# Autodesk Inventor assembly: Leadscrew Bearing Assembly
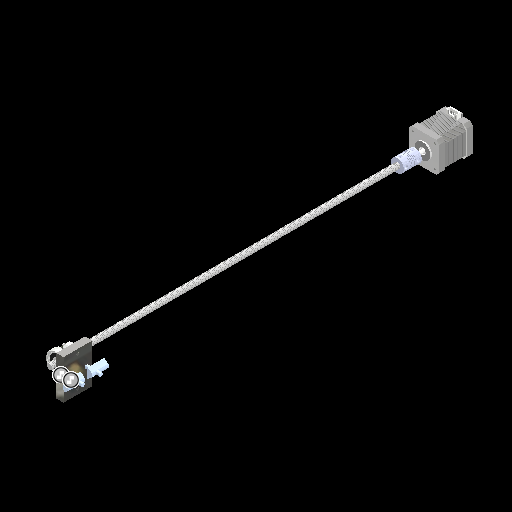
[picture p0: Inventor's stored thumbnail of the model, 512x512]
Saved by Autodesk Inventor 2026.1 (Build 301233000, 233)
## iProperties
Created: 2024-12-30
Part Number: Leadscrew Bearing Assembly
Document SubType Name: Assembly
Designer: drago
Author: drago
## Documents named in this file (9)
- C:\Users\drago\Desktop\_QIST4500_Multidisciplinary_Team_Project\Proteox MX magnet positioner CAD\magnet_positioner_cad_design\z_translator\z_translator.iam
- C:\Users\drago\Desktop\_QIST4500_Multidisciplinary_Team_Project\Proteox MX magnet positioner CAD\magnet_positioner_cad_design\z_translator\5X8_COUPLER.ipt
- C:\Users\drago\Desktop\_QIST4500_Multidisciplinary_Team_Project\Proteox MX magnet positioner CAD\magnet_positioner_cad_design\z_translator\item_61953_t-slot-slider-8-80x40-fa__high.ipt
- C:\Users\drago\Desktop\_QIST4500_Multidisciplinary_Team_Project\Proteox MX magnet positioner CAD\magnet_positioner_cad_design\z_translator\KP08.iam
- C:\Users\drago\Desktop\_QIST4500_Multidisciplinary_Team_Project\Proteox MX magnet positioner CAD\magnet_positioner_cad_design\z_translator\Leadscrew Bearing Bracket.ipt
- C:\Users\drago\Desktop\_QIST4500_Multidisciplinary_Team_Project\Proteox MX magnet positioner CAD\magnet_positioner_cad_design\z_translator\Lead Screw 8mm-2.0 x 500mm.ipt
- C:\Users\drago\Desktop\_QIST4500_Multidisciplinary_Team_Project\Proteox MX magnet positioner CAD\magnet_positioner_cad_design\z_translator\Stepper Motor Nema 17.ipt
- C:\Users\drago\Documents\Inventor\Content Center Files\R2026\en-US\ISO 7089\ISO 7089 - 4 - 140 HV(1).ipt
- C:\Users\drago\Documents\Inventor\Content Center Files\R2026\en-US\ISO 4762(2)\ISO 4762 - M4 x 16ISO.ipt
## Components (11 placed, 8 different names)
1. 5X8_COUPLER:1 — Mate:11, Mate:14, Mate:16, Mate:20
2. item_61953_t-slot-slider-8-80x40-fa__high:1 — Angle:3, Mate:21, Mate:23
3. item_61953_t-slot-slider-8-80x40-fa__high:2 — Angle:2, Mate:22, Mate:24
4. KP08:1 [sub-assembly] — Mate:12, Mate:13, Mate:25, Mate:26, Mate:27, Mate:29, Mate:31
5. Leadscrew Bearing Bracket:1 — Mate:21, Mate:22, Mate:23, Mate:24, Mate:25, Mate:26, Mate:27, Angle:4, Mate:28, Mate:30
6. Lead Screw 8mm-2.0 x 500mm:1 — Mate:11, Mate:12, Mate:13, Mate:15, Mate:19
7. Stepper Motor Nema 17:1 — Mate:14, Mate:15, Mate:16, Mate:17, Mate:18
8. ISO 4762 M4 x 16:2 — Insert:2
9. ISO 7089 4:2 — Mate:30, Mate:31, Insert:2
10. ISO 4762 M4 x 16:1 — Insert:1
11. ISO 7089 4:1 — Mate:28, Mate:29, Insert:1
## Relationships (26: Mate 21, Angle 3, Insert 2)
- Mate:11: 5X8_COUPLER:1 ↔ Lead Screw 8mm-2.0 x 500mm:1
- Mate:12: KP08:1 ↔ Lead Screw 8mm-2.0 x 500mm:1
- Mate:13 (-10 mm): KP08:1 ↔ Lead Screw 8mm-2.0 x 500mm:1
- Mate:14: 5X8_COUPLER:1 ↔ Stepper Motor Nema 17:1
- Mate:15: Lead Screw 8mm-2.0 x 500mm:1 ↔ Stepper Motor Nema 17:1
- Mate:16 (10 mm): 5X8_COUPLER:1 ↔ Stepper Motor Nema 17:1
- Mate:17: Stepper Motor Nema 17:1
- Mate:18: Stepper Motor Nema 17:1
- Mate:19: Lead Screw 8mm-2.0 x 500mm:1
- Angle:2 (0 deg): item_61953_t-slot-slider-8-80x40-fa__high:2
- Angle:3 (180 deg): item_61953_t-slot-slider-8-80x40-fa__high:1
- Mate:20: 5X8_COUPLER:1
- Mate:21: item_61953_t-slot-slider-8-80x40-fa__high:1 ↔ Leadscrew Bearing Bracket:1
- Mate:22: item_61953_t-slot-slider-8-80x40-fa__high:2 ↔ Leadscrew Bearing Bracket:1
- Mate:23: item_61953_t-slot-slider-8-80x40-fa__high:1 ↔ Leadscrew Bearing Bracket:1
- Mate:24: item_61953_t-slot-slider-8-80x40-fa__high:2 ↔ Leadscrew Bearing Bracket:1
- Mate:25: KP08:1 ↔ Leadscrew Bearing Bracket:1
- Mate:26: KP08:1 ↔ Leadscrew Bearing Bracket:1
- Mate:27: KP08:1 ↔ Leadscrew Bearing Bracket:1
- Angle:4 (90 deg): Leadscrew Bearing Bracket:1
- Mate:28: Leadscrew Bearing Bracket:1 ↔ ISO 7089 4:1
- Mate:29: KP08:1 ↔ ISO 7089 4:1
- Insert:1: ISO 4762 M4 x 16:1 ↔ ISO 7089 4:1
- Mate:30: Leadscrew Bearing Bracket:1 ↔ ISO 7089 4:2
- Mate:31: KP08:1 ↔ ISO 7089 4:2
- Insert:2: ISO 4762 M4 x 16:2 ↔ ISO 7089 4:2
